# Autodesk Inventor assembly: Cornerassembly
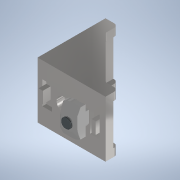
[picture p0: Inventor's stored thumbnail of the model, 180x180]
Saved by Autodesk Inventor 2020.2 (Build 242310000, 310)
## iProperties
Created: 2020-07-25
Part Number: Cornerassembly
Document SubType Name: Assembly
Designer: JK
Author: JK
## Documents named in this file (4)
- C:\Users\JK\Documents\Inventor\Mesa\Cornerassembly.iam
- C:\Users\JK\Documents\Inventor\Mesa\3030cornerbracket.ipt
- C:\Users\JK\Documents\Inventor\Mesa\T_Slot_Nut_Dropin_3030m5ipt.ipt
- C:\Users\JK\Documents\Inventor\Mesa\M5x12BoltFlatHead.ipt
## Components (5 placed, 3 different names)
1. 3030cornerbracket:1 — Mate:3, Angle:1, Mate:4, Mate:5, Mate:6, Angle:2, Mate:7, Mate:8
2. T_Slot_Nut_Dropin_3030m5ipt:1 — Mate:1, Mate:6, Angle:2
3. T_Slot_Nut_Dropin_3030m5ipt:2 — Mate:2, Mate:3, Angle:1
4. M5x12BoltFlatHead:1 — Mate:1, Mate:7, Mate:8
5. M5x12BoltFlatHead:2 — Mate:2, Mate:4, Mate:5
## Relationships (10: Mate 8, Angle 2)
- Mate:1: T_Slot_Nut_Dropin_3030m5ipt:1 ↔ M5x12BoltFlatHead:1
- Mate:2: T_Slot_Nut_Dropin_3030m5ipt:2 ↔ M5x12BoltFlatHead:2
- Mate:3: 3030cornerbracket:1 ↔ T_Slot_Nut_Dropin_3030m5ipt:2
- Angle:1 (0 deg): 3030cornerbracket:1 ↔ T_Slot_Nut_Dropin_3030m5ipt:2
- Mate:4: 3030cornerbracket:1 ↔ M5x12BoltFlatHead:2
- Mate:5: 3030cornerbracket:1 ↔ M5x12BoltFlatHead:2
- Mate:6: 3030cornerbracket:1 ↔ T_Slot_Nut_Dropin_3030m5ipt:1
- Angle:2 (0 deg): 3030cornerbracket:1 ↔ T_Slot_Nut_Dropin_3030m5ipt:1
- Mate:7: 3030cornerbracket:1 ↔ M5x12BoltFlatHead:1
- Mate:8: 3030cornerbracket:1 ↔ M5x12BoltFlatHead:1
